# Autodesk Inventor assembly: 付け根_1
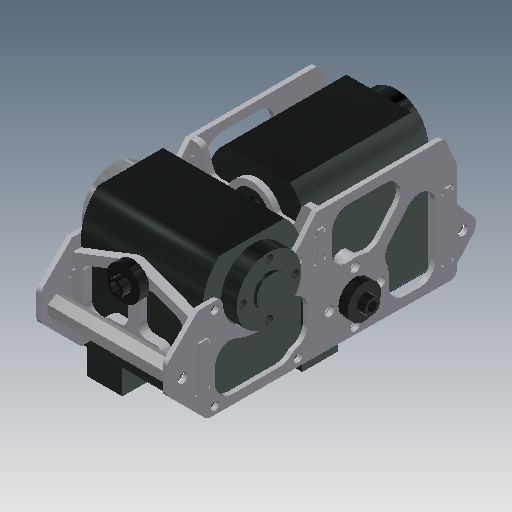
[picture p0: Inventor's stored thumbnail of the model, 512x512]
Saved by Autodesk Inventor 2017.3 (Build 213256000, 256)
## iProperties
Created: 2016-04-27
Part Number: 付け根_1
Document SubType Name: Assembly
Designer: hiroaki
Mass: 257.123 g
Surface Area: 430.699 cm^2
Volume: 127.027 cm^3
Density: 2.02416 g/cm^3
Author: hiroaki
## Documents named in this file (13)
- C:\Users\haya\Desktop\GankenKun0_5\下半身\付け根\付け根_1.iam
- C:\Users\haya\Desktop\GankenKun0_5\既製品\B3M11xx.ipt
- C:\Users\haya\Desktop\GankenKun0_5\既製品\free_horn.ipt
- C:\Users\haya\Desktop\GankenKun0_5\下半身\付け根\付け根_メインフレーム_1_1.ipt
- C:\Users\haya\Desktop\GankenKun0_5\下半身\付け根\付け根_サブフレーム_1_2.ipt
- C:\Users\haya\Desktop\GankenKun0_5\下半身\付け根\付け根_サブフレーム_1_1.ipt
- C:\Users\haya\Desktop\GankenKun0_5\下半身\付け根\付け根_サブフレーム_1_3.ipt
- C:\Users\haya\Desktop\GankenKun0_5\下半身\付け根\付け根_メインフレーム_1_1_MIR.ipt
- C:\Users\haya\Desktop\GankenKun0_5\下半身\リンク\スペーサ\付け根_フリー軸_1_1.ipt
- C:\Users\haya\Desktop\GankenKun0_5\下半身\リンク\スペーサ\付け根_フリー軸_1_2.ipt
- C:\Users\haya\Desktop\GankenKun0_5\下半身\付け根\付け根_サブフレーム_1_4.ipt
- C:\Users\haya\Desktop\GankenKun0_5\既製品\ASU-340.ipt
- C:\Users\haya\Desktop\GankenKun0_5\既製品\CC-0311-08B.ipt
## Components (18 placed, 12 different names)
1. free_horn:1 — 挿入:1
2. B3M11xx:3 — メイト:9, フラッシュ:2, 挿入:1, 挿入:2, 挿入:3, 挿入:4, 挿入:5, 挿入:14, 挿入:15
3. B3M11xx:4 — メイト:9, フラッシュ:2, 挿入:7, 挿入:8, 挿入:9, 挿入:10, 挿入:11, 挿入:12
4. 付け根_メインフレーム_1_1:1 — 挿入:2, 挿入:3, 挿入:4, 挿入:5, メイト:10, メイト:11, メイト:12, メイト:13, メイト:14, メイト:15, メイト:16, メイト:17, 挿入:18, 挿入:19, 挿入:20, 挿入:21, 挿入:29, 挿入:30, 挿入:33
5. 付け根_サブフレーム_1_2:1 — メイト:10, メイト:11, メイト:12, 挿入:7, 挿入:8
6. 付け根_サブフレーム_1_1:1 — 挿入:9, 挿入:10, 挿入:11, 挿入:12, メイト:13, メイト:14
7. 付け根_サブフレーム_1_3:1 — メイト:15, メイト:16, メイト:17, 挿入:36
8. 付け根_メインフレーム_1_1_MIR:1 — 挿入:14, 挿入:15, 挿入:22, 挿入:23, 挿入:24, 挿入:28, 挿入:31, 角度:1, 角度:2, 挿入:35
9. 付け根_フリー軸_1_1:1 — 挿入:18, 挿入:19, 挿入:20, 挿入:21
10. 付け根_フリー軸_1_1:2 — 挿入:22, 挿入:23, 挿入:24
11. 付け根_フリー軸_1_2:1 — 挿入:32
12. 付け根_フリー軸_1_2:2 — 挿入:34
13. 付け根_サブフレーム_1_4:1 — 挿入:37
14. ASU-340:1 — 挿入:28, 挿入:29, 角度:1
15. ASU-340:2 — 挿入:30, 挿入:31, 角度:2
16. CC-0311-08B:1 — 挿入:32, 挿入:33
17. CC-0311-08B:2 — 挿入:34, 挿入:35
18. CC-0311-08B:3 — 挿入:36, 挿入:37
## Relationships (42: Insert 30, Mate 9, Angle 2, Flush 1)
- メイト:9 [Mate]: B3M11xx:3 ↔ B3M11xx:4
- フラッシュ:2 [Flush]: B3M11xx:3 ↔ B3M11xx:4
- 挿入:1 [Insert]: free_horn:1 ↔ B3M11xx:3
- 挿入:2 [Insert]: B3M11xx:3 ↔ 付け根_メインフレーム_1_1:1
- 挿入:3 [Insert]: B3M11xx:3 ↔ 付け根_メインフレーム_1_1:1
- 挿入:4 [Insert]: B3M11xx:3 ↔ 付け根_メインフレーム_1_1:1
- 挿入:5 [Insert]: B3M11xx:3 ↔ 付け根_メインフレーム_1_1:1
- メイト:10 [Mate]: 付け根_メインフレーム_1_1:1 ↔ 付け根_サブフレーム_1_2:1
- メイト:11 [Mate] (0.025 mm): 付け根_メインフレーム_1_1:1 ↔ 付け根_サブフレーム_1_2:1
- メイト:12 [Mate] (0.025 mm): 付け根_メインフレーム_1_1:1 ↔ 付け根_サブフレーム_1_2:1
- 挿入:7 [Insert]: B3M11xx:4 ↔ 付け根_サブフレーム_1_2:1
- 挿入:8 [Insert]: B3M11xx:4 ↔ 付け根_サブフレーム_1_2:1
- 挿入:9 [Insert]: B3M11xx:4 ↔ 付け根_サブフレーム_1_1:1
- 挿入:10 [Insert]: B3M11xx:4 ↔ 付け根_サブフレーム_1_1:1
- 挿入:11 [Insert]: B3M11xx:4 ↔ 付け根_サブフレーム_1_1:1
- 挿入:12 [Insert]: B3M11xx:4 ↔ 付け根_サブフレーム_1_1:1
- メイト:13 [Mate] (0.025 mm): 付け根_メインフレーム_1_1:1 ↔ 付け根_サブフレーム_1_1:1
- メイト:14 [Mate] (0.025 mm): 付け根_メインフレーム_1_1:1 ↔ 付け根_サブフレーム_1_1:1
- メイト:15 [Mate]: 付け根_メインフレーム_1_1:1 ↔ 付け根_サブフレーム_1_3:1
- メイト:16 [Mate] (0.025 mm): 付け根_メインフレーム_1_1:1 ↔ 付け根_サブフレーム_1_3:1
- メイト:17 [Mate] (0.025 mm): 付け根_メインフレーム_1_1:1 ↔ 付け根_サブフレーム_1_3:1
- 挿入:14 [Insert]: B3M11xx:3 ↔ 付け根_メインフレーム_1_1_MIR:1
- 挿入:15 [Insert]: B3M11xx:3 ↔ 付け根_メインフレーム_1_1_MIR:1
- 挿入:18 [Insert]: 付け根_メインフレーム_1_1:1 ↔ 付け根_フリー軸_1_1:1
- 挿入:19 [Insert]: 付け根_メインフレーム_1_1:1 ↔ 付け根_フリー軸_1_1:1
- 挿入:20 [Insert]: 付け根_メインフレーム_1_1:1 ↔ 付け根_フリー軸_1_1:1
- 挿入:21 [Insert]: 付け根_メインフレーム_1_1:1 ↔ 付け根_フリー軸_1_1:1
- 挿入:22 [Insert]: 付け根_メインフレーム_1_1_MIR:1 ↔ 付け根_フリー軸_1_1:2
- 挿入:23 [Insert]: 付け根_メインフレーム_1_1_MIR:1 ↔ 付け根_フリー軸_1_1:2
- 挿入:24 [Insert]: 付け根_メインフレーム_1_1_MIR:1 ↔ 付け根_フリー軸_1_1:2
- 挿入:28 [Insert]: 付け根_メインフレーム_1_1_MIR:1 ↔ ASU-340:1
- 挿入:29 [Insert]: 付け根_メインフレーム_1_1:1 ↔ ASU-340:1
- 挿入:30 [Insert]: 付け根_メインフレーム_1_1:1 ↔ ASU-340:2
- 挿入:31 [Insert]: 付け根_メインフレーム_1_1_MIR:1 ↔ ASU-340:2
- 角度:1 [Angle] (0 deg): 付け根_メインフレーム_1_1_MIR:1 ↔ ASU-340:1
- 角度:2 [Angle] (0 deg): 付け根_メインフレーム_1_1_MIR:1 ↔ ASU-340:2
- 挿入:32 [Insert]: 付け根_フリー軸_1_2:1 ↔ CC-0311-08B:1
- 挿入:33 [Insert]: 付け根_メインフレーム_1_1:1 ↔ CC-0311-08B:1
- 挿入:34 [Insert]: 付け根_フリー軸_1_2:2 ↔ CC-0311-08B:2
- 挿入:35 [Insert]: 付け根_メインフレーム_1_1_MIR:1 ↔ CC-0311-08B:2
- 挿入:36 [Insert]: 付け根_サブフレーム_1_3:1 ↔ CC-0311-08B:3
- 挿入:37 [Insert]: 付け根_サブフレーム_1_4:1 ↔ CC-0311-08B:3
